# Autodesk Inventor assembly: Left XY Drive Mount
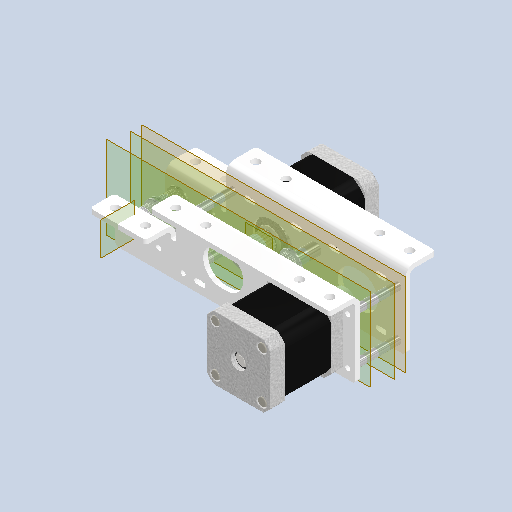
[picture p0: Inventor's stored thumbnail of the model, 512x512]
Saved by Autodesk Inventor 2024 (Build 280153000, 153)
## iProperties
Created: 2024-12-26
Part Number: Left XY Drive Mount
Document SubType Name: Assembly
Designer: Ishaan
Author: Ishaan
## Documents named in this file (10)
- E:\Projects\Axiom--IDEX-3D-Printer\CAD\04 - Gantry\Left XY Drive Mount.iam
- E:\Projects\Axiom--IDEX-3D-Printer\CAD\04 - Gantry\XY Motor Mount A.ipt
- E:\Projects\Axiom--IDEX-3D-Printer\CAD\04 - Gantry\XY Motor Mount B.ipt
- E:\Projects\Axiom--IDEX-3D-Printer\CAD\00 - COTS Components\Hardware\M3 30mm Standoff.ipt
- E:\Projects\Axiom--IDEX-3D-Printer\CAD\00 - COTS Components\NEMA 17 - Long\NEMA 17 Long.ipt
- E:\Projects\Axiom--IDEX-3D-Printer\CAD\00 - COTS Components\10mm 20T GT2 Timing Pulley 5mm Bore\10mm 20T GT2 Timing Pulley 5mm Bore.ipt
- E:\Projects\Axiom--IDEX-3D-Printer\CAD\00 - COTS Components\Hardware\M5 Shim 0p5mm.ipt
- E:\Projects\Axiom--IDEX-3D-Printer\CAD\00 - COTS Components\10mm 20T GT2 Idler Pulley 5mm Bore\10mm 20T GT2 Idler Pulley 5mm Bore.ipt
- E:\Projects\Axiom--IDEX-3D-Printer\CAD\00 - COTS Components\10mm Smooth Idler Pulley 5mm Bore\10mm 20T Smooth Idler Pulley 5mm Bore.ipt
- E:\Projects\Axiom--IDEX-3D-Printer\CAD\00 - COTS Components\Hardware\M5 Spacer 15mm.ipt
## Components (30 placed, 9 different names)
1. XY Motor Mount A:1 — Insert:1, Insert:2, Insert:3, Insert:4, Insert:5, Insert:6, Insert:7, Insert:8, Flush:3, Insert:19, Insert:20, Insert:21, Insert:22, Insert:31, Insert:32, Symmetry:1
2. XY Motor Mount B:1 — Insert:9, Insert:10, Insert:11, Insert:12, Insert:13, Insert:14, Insert:15, Insert:16, Flush:1, Insert:17, Insert:18, Insert:23, Insert:24, Insert:35, Insert:36, Symmetry:1
3. NEMA 17 Long:1 — Mate:1, Insert:17, Insert:18, Angle:1
4. NEMA 17 Long:2 — Mate:2, Insert:19, Insert:20, Angle:2
5. 10mm 20T GT2 Timing Pulley 5mm Bore:1 — Flush:2, Mate:1, Angle:1
6. 10mm 20T GT2 Timing Pulley 5mm Bore:2 — Flush:4, Mate:2, Angle:2
7. M5 Shim 0p5mm:1 — Insert:30
8. 10mm 20T GT2 Idler Pulley 5mm Bore:1 — Insert:28
9. 10mm 20T GT2 Idler Pulley 5mm Bore:2 — Insert:27, Insert:29
10. 10mm 20T Smooth Idler Pulley 5mm Bore:1 — Insert:25, Insert:30
11. 10mm 20T Smooth Idler Pulley 5mm Bore:2 — Insert:26
12. 10mm 20T GT2 Idler Pulley 5mm Bore:3 — Insert:33
13. 10mm 20T GT2 Idler Pulley 5mm Bore:4 — Insert:34
14. M3 30mm Standoff:1 — Insert:1, Insert:9
15. M3 30mm Standoff:2 — Insert:2, Insert:10
16. M3 30mm Standoff:3 — Insert:3, Insert:12
17. M3 30mm Standoff:4 — Insert:4, Insert:11
18. M3 30mm Standoff:5 — Insert:5, Insert:14
19. M3 30mm Standoff:6 — Insert:6, Insert:13
20. M3 30mm Standoff:7 — Insert:7, Insert:16
21. M3 30mm Standoff:8 — Insert:8, Insert:15
22. M5 Shim 0p5mm:7 — Insert:31, Insert:34
23. M5 Shim 0p5mm:8 — Insert:32, Insert:33
24. M5 Spacer 15mm:1 — Insert:35
25. M5 Spacer 15mm:2 — Insert:36
26. M5 Shim 0p5mm:2 — Insert:29
27. M5 Shim 0p5mm:3 — Insert:24, Insert:25
28. M5 Shim 0p5mm:4 — Insert:23, Insert:27
29. M5 Shim 0p5mm:5 — Insert:22, Insert:28
30. M5 Shim 0p5mm:6 — Insert:21, Insert:26
## Relationships (45: Insert 36, Flush 4, Mate 2, Angle 2, Symmetry 1)
- Insert:1: XY Motor Mount A:1 ↔ M3 30mm Standoff:1
- Insert:2: XY Motor Mount A:1 ↔ M3 30mm Standoff:2
- Insert:3: XY Motor Mount A:1 ↔ M3 30mm Standoff:3
- Insert:4: XY Motor Mount A:1 ↔ M3 30mm Standoff:4
- Insert:5: XY Motor Mount A:1 ↔ M3 30mm Standoff:5
- Insert:6: XY Motor Mount A:1 ↔ M3 30mm Standoff:6
- Insert:7: XY Motor Mount A:1 ↔ M3 30mm Standoff:7
- Insert:8: XY Motor Mount A:1 ↔ M3 30mm Standoff:8
- Insert:9: XY Motor Mount B:1 ↔ M3 30mm Standoff:1
- Insert:10: XY Motor Mount B:1 ↔ M3 30mm Standoff:2
- Insert:11: XY Motor Mount B:1 ↔ M3 30mm Standoff:4
- Insert:12: XY Motor Mount B:1 ↔ M3 30mm Standoff:3
- Insert:13: XY Motor Mount B:1 ↔ M3 30mm Standoff:6
- Insert:14: XY Motor Mount B:1 ↔ M3 30mm Standoff:5
- Insert:15: XY Motor Mount B:1 ↔ M3 30mm Standoff:8
- Insert:16: XY Motor Mount B:1 ↔ M3 30mm Standoff:7
- Flush:1 (7.5 mm): XY Motor Mount B:1
- Flush:2: 10mm 20T GT2 Timing Pulley 5mm Bore:1
- Mate:1: NEMA 17 Long:1 ↔ 10mm 20T GT2 Timing Pulley 5mm Bore:1
- Insert:17: XY Motor Mount B:1 ↔ NEMA 17 Long:1
- Insert:18: XY Motor Mount B:1 ↔ NEMA 17 Long:1
- Angle:1 (0 deg): NEMA 17 Long:1 ↔ 10mm 20T GT2 Timing Pulley 5mm Bore:1
- Flush:3 (7.5 mm): XY Motor Mount A:1
- Flush:4: 10mm 20T GT2 Timing Pulley 5mm Bore:2
- Mate:2: NEMA 17 Long:2 ↔ 10mm 20T GT2 Timing Pulley 5mm Bore:2
- Insert:19: XY Motor Mount A:1 ↔ NEMA 17 Long:2
- Insert:20: XY Motor Mount A:1 ↔ NEMA 17 Long:2
- Angle:2 (0 deg): NEMA 17 Long:2 ↔ 10mm 20T GT2 Timing Pulley 5mm Bore:2
- Insert:21: XY Motor Mount A:1 ↔ M5 Shim 0p5mm:6
- Insert:22: XY Motor Mount A:1 ↔ M5 Shim 0p5mm:5
- Insert:23: XY Motor Mount B:1 ↔ M5 Shim 0p5mm:4
- Insert:24: XY Motor Mount B:1 ↔ M5 Shim 0p5mm:3
- Insert:25: 10mm 20T Smooth Idler Pulley 5mm Bore:1 ↔ M5 Shim 0p5mm:3
- Insert:26: 10mm 20T Smooth Idler Pulley 5mm Bore:2 ↔ M5 Shim 0p5mm:6
- Insert:27: 10mm 20T GT2 Idler Pulley 5mm Bore:2 ↔ M5 Shim 0p5mm:4
- Insert:28: 10mm 20T GT2 Idler Pulley 5mm Bore:1 ↔ M5 Shim 0p5mm:5
- Insert:29: 10mm 20T GT2 Idler Pulley 5mm Bore:2 ↔ M5 Shim 0p5mm:2
- Insert:30: M5 Shim 0p5mm:1 ↔ 10mm 20T Smooth Idler Pulley 5mm Bore:1
- Insert:31: XY Motor Mount A:1 ↔ M5 Shim 0p5mm:7
- Insert:32: XY Motor Mount A:1 ↔ M5 Shim 0p5mm:8
- Insert:33: 10mm 20T GT2 Idler Pulley 5mm Bore:3 ↔ M5 Shim 0p5mm:8
- Insert:34: 10mm 20T GT2 Idler Pulley 5mm Bore:4 ↔ M5 Shim 0p5mm:7
- Insert:35: XY Motor Mount B:1 ↔ M5 Spacer 15mm:1
- Insert:36: XY Motor Mount B:1 ↔ M5 Spacer 15mm:2
- Symmetry:1: XY Motor Mount A:1 ↔ XY Motor Mount B:1
